# Autodesk Inventor assembly: Assembly1
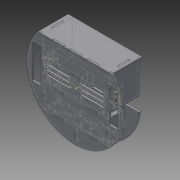
[picture p0: Inventor's stored thumbnail of the model, 180x180]
Saved by Autodesk Inventor 2015 (Build 190159000, 159)
## iProperties
Created: 2014-08-15
Part Number: Assembly1
Document SubType Name: Assembly
Designer: karl
Author: karl
## Documents named in this file (10)
- C:\Users\karl\Documents\GitHub\SUMOChassis\Body\Assembly1.iam
- C:\Users\karl\Documents\GitHub\SUMOChassis\Body\BasePlate.ipt
- C:\Users\karl\Documents\GitHub\SUMOChassis\Body\Motor support.ipt
- C:\Users\karl\Documents\GitHub\SUMOChassis\Body\Frount plate.ipt
- C:\Users\karl\Documents\GitHub\SUMOChassis\Body\motor reinforcment.ipt
- C:\Users\karl\Documents\GitHub\SUMOChassis\Body\Standard Parts\Motor.ipt
- C:\Users\karl\Documents\GitHub\SUMOChassis\Body\Battery holder.ipt
- C:\Users\karl\Documents\GitHub\SUMOChassis\Body\battery holder ends.ipt
- C:\Users\karl\Documents\GitHub\SUMOChassis\Body\Back support.ipt
- C:\Users\karl\Documents\GitHub\SUMOChassis\Body\Mid Plate.ipt
## Components (13 placed, 9 different names)
1. BasePlate:1 — Flush:1, Flush:2, Flush:3, Flush:5, Flush:7, Flush:9, Mate:6, Mate:7, Mate:8, Flush:16, Flush:22, Mate:11, Mate:13
2. Motor support:1 — Flush:1, Flush:2, Flush:3, Flush:4, Mate:1, Flush:6, Mate:2, Mate:3, Mate:4, Mate:5
3. Frount plate:1 — Flush:4, Flush:5, Mate:1, Flush:15, Flush:17
4. motor reinforcment:1 — Flush:6, Mate:2, Flush:7
5. Motor:1 — Mate:3, Mate:4, Mate:5, Mate:9, Flush:21
6. Battery holder:1 — Flush:9, Mate:6, Mate:7, Flush:10, Flush:11
7. Battery holder:2 — Flush:10, Flush:11, Mate:8, Flush:12, Flush:13, Flush:14, Flush:18, Flush:19, Flush:20, Flush:23
8. battery holder ends:1 — Flush:12, Flush:13, Flush:14
9. Motor support:2 — Flush:15, Flush:16, Flush:17, Mate:10, Mate:12
10. battery holder ends:2 — Flush:18, Flush:19, Flush:20
11. Motor:2 — Mate:9, Mate:10, Flush:21
12. Back support:1 — Flush:22, Flush:23, Mate:11, Mate:14
13. Mid Plate:1 — Mate:12, Mate:13, Mate:14
## Relationships (36: Flush 22, Mate 14)
- Flush:1: BasePlate:1 ↔ Motor support:1
- Flush:2: BasePlate:1 ↔ Motor support:1
- Flush:3: BasePlate:1 ↔ Motor support:1
- Flush:4: Motor support:1 ↔ Frount plate:1
- Flush:5: BasePlate:1 ↔ Frount plate:1
- Mate:1: Motor support:1 ↔ Frount plate:1
- Flush:6: Motor support:1 ↔ motor reinforcment:1
- Mate:2: Motor support:1 ↔ motor reinforcment:1
- Flush:7: BasePlate:1 ↔ motor reinforcment:1
- Mate:3: Motor support:1 ↔ Motor:1
- Mate:4: Motor support:1 ↔ Motor:1
- Mate:5: Motor support:1 ↔ Motor:1
- Flush:9: BasePlate:1 ↔ Battery holder:1
- Mate:6: BasePlate:1 ↔ Battery holder:1
- Mate:7: BasePlate:1 ↔ Battery holder:1
- Flush:10: Battery holder:1 ↔ Battery holder:2
- Flush:11: Battery holder:1 ↔ Battery holder:2
- Mate:8: BasePlate:1 ↔ Battery holder:2
- Flush:12: Battery holder:2 ↔ battery holder ends:1
- Flush:13: Battery holder:2 ↔ battery holder ends:1
- Flush:14: Battery holder:2 ↔ battery holder ends:1
- Flush:15: Frount plate:1 ↔ Motor support:2
- Flush:16: BasePlate:1 ↔ Motor support:2
- Flush:17: Frount plate:1 ↔ Motor support:2
- Flush:18: Battery holder:2 ↔ battery holder ends:2
- Flush:19: Battery holder:2 ↔ battery holder ends:2
- Flush:20: Battery holder:2 ↔ battery holder ends:2
- Mate:9: Motor:1 ↔ Motor:2
- Mate:10: Motor support:2 ↔ Motor:2
- Flush:21: Motor:1 ↔ Motor:2
- Flush:22: BasePlate:1 ↔ Back support:1
- Flush:23: Battery holder:2 ↔ Back support:1
- Mate:11: BasePlate:1 ↔ Back support:1
- Mate:12: Motor support:2 ↔ Mid Plate:1
- Mate:13: BasePlate:1 ↔ Mid Plate:1
- Mate:14: Back support:1 ↔ Mid Plate:1
